# Autodesk Inventor assembly: curve_module_test
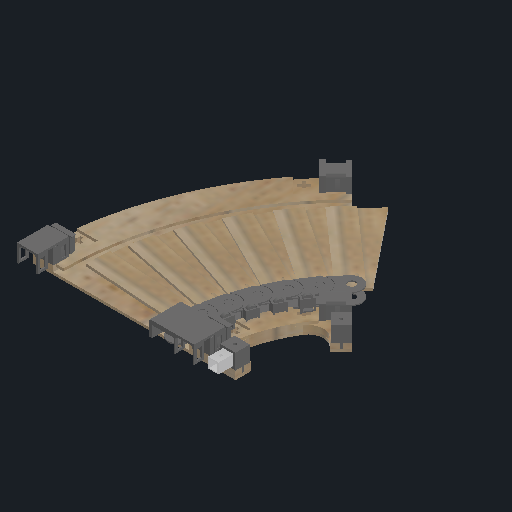
[picture p0: Inventor's stored thumbnail of the model, 512x512]
Saved by Autodesk Inventor 2026.1 (Build 301233020, 233B)
## iProperties
Created: 2025-09-28
Part Number: curve_module_test
Document SubType Name: Assembly
Designer: hibik
Author: hibik
## Documents named in this file (6)
- C:\Users\hibik\Documents\Robomech\conveyer\curve_module\curve_module_test.iam
- C:\Users\hibik\Documents\Robomech\conveyer\curve_module\Assy_curve_module.iam
- C:\Users\hibik\Documents\Robomech\conveyer\belt\belt_curve.iam
- C:\Users\hibik\Documents\Robomech\conveyer\connector_module\connetcor_female.ipt
- C:\Users\hibik\Documents\Robomech\conveyer\connector_module\connetcor_female_cover.ipt
- C:\Users\hibik\Documents\Robomech\conveyer\connector_module\position_setter_bar.ipt
## Components (5 placed, 5 different names)
1. Assy_curve_module:1 [sub-assembly] — 正接:1, メイト:1, 角度:1, 正接:2, メイト:2, メイト:3, メイト:4, メイト:5, メイト:6, メイト:7, メイト:8, メイト:9, フラッシュ:1
2. belt_curve:1 [sub-assembly] — 正接:1, メイト:1, 角度:1, 正接:2
3. connetcor_female:1 — メイト:2, メイト:3, メイト:4
4. connetcor_female_cover:1 — メイト:5, メイト:6, メイト:7
5. position_setter_bar:1 — メイト:8, メイト:9, フラッシュ:1
## Relationships (13: Mate 9, Tangent 2, Angle 1, Flush 1)
- 正接:1 [Tangent]: Assy_curve_module:1 ↔ belt_curve:1
- メイト:1 [Mate]: Assy_curve_module:1 ↔ belt_curve:1
- 角度:1 [Angle] (-3.75 deg): Assy_curve_module:1 ↔ belt_curve:1
- 正接:2 [Tangent]: Assy_curve_module:1 ↔ belt_curve:1
- メイト:2 [Mate] (0.5 mm): Assy_curve_module:1 ↔ connetcor_female:1
- メイト:3 [Mate] (0.5 mm): Assy_curve_module:1 ↔ connetcor_female:1
- メイト:4 [Mate] (0.6 mm): Assy_curve_module:1 ↔ connetcor_female:1
- メイト:5 [Mate] (0.5 mm): Assy_curve_module:1 ↔ connetcor_female_cover:1
- メイト:6 [Mate] (0.5 mm): Assy_curve_module:1 ↔ connetcor_female_cover:1
- メイト:7 [Mate] (0.6 mm): Assy_curve_module:1 ↔ connetcor_female_cover:1
- メイト:8 [Mate] (0.5 mm): Assy_curve_module:1 ↔ position_setter_bar:1
- メイト:9 [Mate] (0.5 mm): Assy_curve_module:1 ↔ position_setter_bar:1
- フラッシュ:1 [Flush]: Assy_curve_module:1 ↔ position_setter_bar:1
